# Autodesk Inventor assembly: bit-bot assembly
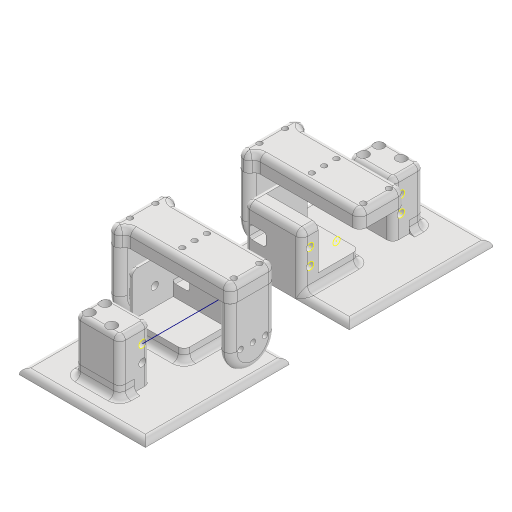
[picture p0: Inventor's stored thumbnail of the model, 512x512]
Saved by Autodesk Inventor 2024 (Build 280153000, 153)
## iProperties
Created: 2024-01-21
Part Number: bit-bot assembly
Document SubType Name: Assembly
Designer: chris
Author: chris
## Documents named in this file (9)
- C:\Users\chris\Desktop\STL files\bit-bot\bit-bot assembly.iam
- C:\Users\chris\Desktop\STL files\bit-bot\left foot link.ipt
- C:\Users\chris\Desktop\STL files\bit-bot\ball bearing holder smoltronv2.ipt
- C:\Users\chris\Desktop\STL files\bit-bot\connecting plate servo flat v5.ipt
- C:\Users\chris\Desktop\STL files\bit-bot\servo horn holder smoltronv2.ipt
- C:\Users\chris\Desktop\STL files\bit-bot\right_foot_smoltron.ipt
- C:\Users\chris\Desktop\STL files\bit-bot\right foot link.ipt
- C:\Users\chris\Desktop\STL files\bit-bot\left_foot_smoltron.ipt
- C:\Users\chris\Desktop\STL files\bit-bot\ball bearing connector.ipt
## Components (12 placed, 8 different names)
1. left foot link:1 — Rigid:7
2. ball bearing holder smoltronv2:1 — Rigid:3, Rigid:8, Rotational:5
3. connecting plate servo flat v5:1 — Rigid:3, Rigid:4
4. servo horn holder smoltronv2:1 — Rigid:4
5. right_foot_smoltron:1 — Rotational:1, Rigid:6, Flush:1, Mate:1
6. right foot link:1 — Rotational:1
7. ball bearing holder smoltronv2:2 — Rigid:6, Rigid:5, Rotational:6
8. connecting plate servo flat v5:2 — Rigid:5, Rotational:3, Rotational:4
9. servo horn holder smoltronv2:2 — Rotational:3, Rotational:4
10. left_foot_smoltron:1 — Flush:1, Rigid:7, Rigid:8, Mate:1
11. ball bearing connector:1 — Rotational:6
12. ball bearing connector:2 — Rotational:5
## Relationships (13: WeldJoint 6, RevoluteJoint 5, Flush 1, Mate 1)
- Rigid:3 [WeldJoint]: ball bearing holder smoltronv2:1 ↔ connecting plate servo flat v5:1
- Rigid:4 [WeldJoint]: connecting plate servo flat v5:1 ↔ servo horn holder smoltronv2:1
- Rotational:1 [RevoluteJoint]: right_foot_smoltron:1 ↔ right foot link:1
- Rigid:6 [WeldJoint]: right_foot_smoltron:1 ↔ ball bearing holder smoltronv2:2
- Rigid:5 [WeldJoint]: ball bearing holder smoltronv2:2 ↔ connecting plate servo flat v5:2
- Rotational:3 [RevoluteJoint]: connecting plate servo flat v5:2 ↔ servo horn holder smoltronv2:2
- Rotational:4 [RevoluteJoint]: connecting plate servo flat v5:2 ↔ servo horn holder smoltronv2:2
- Flush:1: right_foot_smoltron:1 ↔ left_foot_smoltron:1
- Rigid:7 [WeldJoint]: left foot link:1 ↔ left_foot_smoltron:1
- Rigid:8 [WeldJoint]: ball bearing holder smoltronv2:1 ↔ left_foot_smoltron:1
- Rotational:5 [RevoluteJoint]: ball bearing holder smoltronv2:1 ↔ ball bearing connector:2
- Rotational:6 [RevoluteJoint]: ball bearing holder smoltronv2:2 ↔ ball bearing connector:1
- Mate:1: right_foot_smoltron:1 ↔ left_foot_smoltron:1
